# Autodesk Inventor assembly: aio_head_part
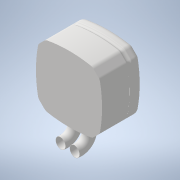
[picture p0: Inventor's stored thumbnail of the model, 180x180]
Saved by Autodesk Inventor 2022 (Build 260153000, 153)
## iProperties
Created: 2021-05-19
Part Number: aio_head_part
Document SubType Name: Assembly
Designer: 6128059
Author: 6128059
## Documents named in this file (3)
- C:\Users\sbbgi\Documents\GitHub\eatx_case\atx\resources\aio-cooler-1.snapshot.2\AIO Cooler\aio_head_part.iam
- C:\Users\sbbgi\Documents\GitHub\eatx_case\atx\resources\aio-cooler-1.snapshot.2\AIO Cooler\Water block.ipt
- C:\Users\sbbgi\Documents\GitHub\eatx_case\atx\resources\aio-cooler-1.snapshot.2\AIO Cooler\Rørende - water block.ipt
## Components (3 placed, 2 different names)
1. Water block:1 — Mate:24, Mate:25, Mate:26, Mate:27
2. Rørende - water block:1 — Mate:25, Mate:27, Angle:1
3. Rørende - water block:2 — Mate:24, Mate:26, Angle:1
## Relationships (5: Mate 4, Angle 1)
- Mate:24: Water block:1 ↔ Rørende - water block:2
- Mate:25: Water block:1 ↔ Rørende - water block:1
- Mate:26: Water block:1 ↔ Rørende - water block:2
- Mate:27: Water block:1 ↔ Rørende - water block:1
- Angle:1 (0 deg): Rørende - water block:1 ↔ Rørende - water block:2
